# Autodesk Inventor assembly: GTPR Assembly - Laci
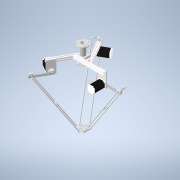
[picture p0: Inventor's stored thumbnail of the model, 180x180]
Saved by Autodesk Inventor 2021 (Build 250183000, 183)
## iProperties
Created: 2022-09-08
Part Number: GTPR Assembly - Laci
Document SubType Name: Assembly
Designer: Administrator
Title: GTPR Assembly - Laci v13
Author: Administrator
## Documents named in this file (17)
- C:\Git\PhD\Inventor\GTPR_toBeBuilt\GTPR Assembly - Laci.iam
- C:\Git\PhD\Inventor\GTPR_toBeBuilt\base frame.iam
- C:\Git\PhD\Inventor\GTPR_toBeBuilt\motor shaft clamp.ipt
- C:\Git\PhD\Inventor\GTPR_toBeBuilt\bosch b6 20x20 250 v1.ipt
- C:\Git\PhD\Inventor\GTPR_toBeBuilt\elbow keeper v1.ipt
- C:\Git\PhD\Inventor\GTPR_toBeBuilt\M8 Nut v5 v1.ipt
- C:\Git\PhD\Inventor\GTPR_toBeBuilt\inner.ipt
- C:\Git\PhD\Inventor\GTPR_toBeBuilt\outer.ipt
- C:\Git\PhD\Inventor\GTPR_toBeBuilt\lower arm 800.ipt
- C:\Git\PhD\Inventor\GTPR_toBeBuilt\WorkTriangleDisk.ipt
- C:\Git\PhD\Inventor\GTPR_toBeBuilt\workTrianglePc1.ipt
- C:\Users\szucs\Documents\Inventor\Content Center Files\R2021\en-US\AS 1420\AS 1420 - 1973 - M4 x 20.ipt
- C:\Users\szucs\Documents\Inventor\Content Center Files\R2021\en-US\AS 1237 (2.1)\AS 1237 - 4.ipt
- C:\Git\PhD\Inventor\GTPR_toBeBuilt\SKF_CAD_MODEL_SKF_W 624 R\AIS2021\SKF_W 624 R.iam
- C:\Git\PhD\Inventor\GTPR_toBeBuilt\rodFixerWasher.ipt
- C:\Git\PhD\Inventor\GTPR_toBeBuilt\rodFixer.ipt
- C:\Git\PhD\Inventor\GTPR_toBeBuilt\elbow clamp.ipt
## Components (95 placed, 16 different names)
1. base frame:1 [sub-assembly] — Flush:27, Mate:260, Flush:28, Mate:261, Flush:29, Mate:262, Angle:11, Angle:12, Angle:13
2. bosch b6 20x20 250 v1:2 — Mate:265, Flush:34, Flush:35, Flush:40, Flush:41, Mate:268
3. bosch b6 20x20 250 v1:3 — Flush:30, Flush:31, Mate:263, Flush:36, Flush:37, Mate:266
4. bosch b6 20x20 250 v1:4 — Mate:264, Flush:32, Flush:33, Flush:38, Mate:267, Flush:39
5. elbow keeper v1:1 — Mate:37, Mate:38, Flush:21, Flush:23, Mate:47, Mate:67, Mate:68, Mate:93, Mate:94, Mate:277
6. elbow keeper v1:2 — Mate:39, Mate:40, Flush:20, Flush:22, Mate:44, Mate:69, Mate:70, Mate:95, Mate:96, Mate:269
7. elbow keeper v1:3 — Mate:41, Mate:42, Flush:18, Flush:19, Mate:45, Mate:71, Mate:72, Mate:91, Mate:92, Mate:273
8. M8 Nut v5 v1:1 — Mate:38, Flush:21, Mate:196
9. M8 Nut v5 v1:2 — Mate:37, Flush:23, Mate:197
10. M8 Nut v5 v1:3 — Mate:39, Flush:20, Mate:198
11. M8 Nut v5 v1:4 — Mate:42, Flush:18, Mate:195
12. M8 Nut v5 v1:5 — Mate:40, Flush:22, Mate:199
13. M8 Nut v5 v1:6 — Mate:41, Flush:19, Mate:194
14. M8 Nut v5 v1:7 — Mate:44, Mate:270
15. M8 Nut v5 v1:9 — Mate:45, Mate:275
16. M8 Nut v5 v1:10 — Mate:47, Mate:279
17. inner:1 — Mate:72, Tangent:3, Mate:101, Mate:195
18. inner:2 — Mate:71, Tangent:4, Mate:102, Mate:194
19. inner:3 — Mate:70, Tangent:5, Mate:97, Mate:199
20. inner:4 — Mate:69, Tangent:6, Mate:98, Mate:198
21. inner:5 — Mate:68, Tangent:1, Mate:100, Mate:197
22. inner:6 — Mate:67, Tangent:2, Mate:99, Mate:196
23. outer:1 — Tangent:6, Mate:81, Mate:82
24. outer:2 — Tangent:5, Mate:79, Mate:80
25. outer:3 — Tangent:1, Mate:84, Mate:85
26. outer:4 — Tangent:2, Mate:83, Mate:86
27. outer:5 — Tangent:4, Mate:87, Mate:90
28. outer:6 — Tangent:3, Mate:88, Mate:89
29. lower arm 800:1 — Mate:79, Mate:80, Mate:123, Mate:124, Angle:10, Tangent:15, Mate:202
30. lower arm 800:2 — Mate:81, Mate:82, Mate:122, Mate:125, Angle:9, Mate:201, Tangent:14
31. lower arm 800:3 — Mate:84, Mate:85, Mate:119, Mate:158, Angle:8, Mate:259
32. lower arm 800:4 — Mate:83, Mate:86, Mate:120, Mate:121, Angle:7, Mate:258, Tangent:17
33. lower arm 800:5 — Mate:87, Mate:90, Mate:116, Mate:117, Angle:6, Mate:256, Tangent:16
34. lower arm 800:6 — Mate:88, Mate:89, Mate:115, Mate:118, Angle:5, Mate:257
35. M8 Nut v5 v1:13 — Mate:91, Mate:101, Mate:282
36. M8 Nut v5 v1:14 — Mate:96, Mate:98
37. M8 Nut v5 v1:15 — Mate:95, Mate:97, Mate:281
38. M8 Nut v5 v1:16 — Mate:93, Mate:100
39. M8 Nut v5 v1:17 — Mate:92, Mate:102
40. M8 Nut v5 v1:18 — Mate:94, Mate:99, Mate:283
41. inner:7 — Tangent:11, Mate:209, Mate:210
42. inner:8 — Tangent:12, Mate:207, Mate:208
43. inner:9 — Tangent:9, Mate:203, Mate:204
44. inner:10 — Tangent:10, Mate:205, Mate:206
45. inner:11 — Tangent:8, Mate:150, Mate:152
46. inner:12 — Tangent:13, Mate:151, Mate:153
47. outer:7 — Tangent:12, Mate:119, Mate:158, Angle:8
48. outer:8 — Tangent:11, Mate:120, Mate:121, Angle:7
49. outer:9 — Tangent:10, Mate:115, Mate:118, Angle:5
50. outer:10 — Tangent:9, Mate:116, Mate:117, Angle:6
51. outer:11 — Mate:123, Mate:124, Tangent:13, Angle:10
52. outer:12 — Tangent:8, Mate:122, Mate:125, Angle:9
53. WorkTriangleDisk:1 — Mate:284, Mate:285, Mate:286, Mate:287, Mate:288, Mate:289, Mate:290, Mate:291, Mate:292, Mate:293, Mate:294, Mate:295
54. workTrianglePc1:3 — Mate:207, Mate:208, Mate:209, Mate:210, Mate:286, Mate:287, Mate:292, Mate:293
55. workTrianglePc1:4 — Mate:203, Mate:204, Mate:205, Mate:206, Mate:285, Mate:288, Mate:289, Mate:294
56. workTrianglePc1:5 — Mate:150, Mate:151, Mate:152, Mate:153, Mate:284, Mate:290, Mate:291, Mate:295
57. AS 1420 - Metric M4 x 20:1 — Mate:171, Mate:174, Mate:177, Mate:178, Mate:200, Mate:202
58. AS 1237 (2.1) 4:3 — Mate:170, Mate:200, Tangent:15
59. SKF_W 624 R:1 [sub-assembly] — Mate:170, Mate:171, Mate:175, Mate:212, Mate:213
60. AS 1237 (2.1) 4:4 — Mate:174, Mate:175, Mate:176
61. rodFixerWasher:1 — Mate:176, Mate:177, Mate:178, Flush:24
62. AS 1420 - Metric M4 x 20:2 — Mate:183, Mate:184, Mate:186, Mate:188, Mate:189, Mate:201
63. AS 1237 (2.1) 4:5 — Mate:189, Tangent:14
64. SKF_W 624 R:2 [sub-assembly] — Mate:187, Mate:188, Mate:211
65. AS 1237 (2.1) 4:6 — Mate:185, Mate:186, Mate:187
66. rodFixerWasher:2 — Mate:183, Mate:184, Mate:185, Flush:24
67. rodFixer:1 — Mate:211, Mate:212, Mate:213
68. AS 1420 - Metric M4 x 20:3 — Mate:256
69. AS 1237 (2.1) 4:7 — Tangent:16
70. SKF_W 624 R:3 [sub-assembly]
71. AS 1237 (2.1) 4:8
72. rodFixerWasher:3
73. AS 1420 - Metric M4 x 20:4 — Mate:257
74. AS 1237 (2.1) 4:9
75. SKF_W 624 R:4 [sub-assembly]
76. AS 1237 (2.1) 4:10
77. rodFixerWasher:4
78. rodFixer:2
79. AS 1420 - Metric M4 x 20:5 — Mate:259
80. AS 1237 (2.1) 4:11
81. SKF_W 624 R:5 [sub-assembly]
82. AS 1237 (2.1) 4:12
83. rodFixerWasher:5
84. AS 1420 - Metric M4 x 20:6 — Mate:258
85. AS 1237 (2.1) 4:13 — Tangent:17
86. SKF_W 624 R:6 [sub-assembly]
87. AS 1237 (2.1) 4:14
88. rodFixerWasher:6
89. rodFixer:3
90. motor shaft clamp:1 — Flush:27, Mate:260, Mate:265, Flush:34, Flush:35, Angle:11
91. motor shaft clamp:2 — Flush:29, Mate:262, Flush:30, Flush:31, Mate:263, Angle:12
92. motor shaft clamp:3 — Flush:28, Mate:261, Mate:264, Flush:32, Flush:33, Angle:13
93. elbow clamp:1 — Flush:36, Flush:37, Mate:266, Mate:273, Mate:275, Mate:282
94. elbow clamp:2 — Flush:38, Mate:267, Flush:39, Mate:269, Mate:270, Mate:281
95. elbow clamp:3 — Flush:40, Flush:41, Mate:268, Mate:277, Mate:279, Mate:283
## Relationships (217: Mate 168, Flush 24, Tangent 16, Angle 9)
- Mate:37: elbow keeper v1:1 ↔ M8 Nut v5 v1:2
- Mate:38: elbow keeper v1:1 ↔ M8 Nut v5 v1:1
- Mate:39: elbow keeper v1:2 ↔ M8 Nut v5 v1:3
- Mate:40: elbow keeper v1:2 ↔ M8 Nut v5 v1:5
- Mate:41: elbow keeper v1:3 ↔ M8 Nut v5 v1:6
- Mate:42: elbow keeper v1:3 ↔ M8 Nut v5 v1:4
- Flush:18: elbow keeper v1:3 ↔ M8 Nut v5 v1:4
- Flush:19: elbow keeper v1:3 ↔ M8 Nut v5 v1:6
- Flush:20: elbow keeper v1:2 ↔ M8 Nut v5 v1:3
- Flush:21: elbow keeper v1:1 ↔ M8 Nut v5 v1:1
- Flush:22: elbow keeper v1:2 ↔ M8 Nut v5 v1:5
- Flush:23: elbow keeper v1:1 ↔ M8 Nut v5 v1:2
- Mate:44: elbow keeper v1:2 ↔ M8 Nut v5 v1:7
- Mate:45: elbow keeper v1:3 ↔ M8 Nut v5 v1:9
- Mate:47: elbow keeper v1:1 ↔ M8 Nut v5 v1:10
- Mate:67: elbow keeper v1:1 ↔ inner:6
- Mate:68: elbow keeper v1:1 ↔ inner:5
- Mate:69: elbow keeper v1:2 ↔ inner:4
- Mate:70: elbow keeper v1:2 ↔ inner:3
- Mate:71: elbow keeper v1:3 ↔ inner:2
- Mate:72: elbow keeper v1:3 ↔ inner:1
- Tangent:1: inner:5 ↔ outer:3
- Tangent:2: inner:6 ↔ outer:4
- Tangent:3: inner:1 ↔ outer:6
- Tangent:4: inner:2 ↔ outer:5
- Tangent:5: inner:3 ↔ outer:2
- Tangent:6: inner:4 ↔ outer:1
- Mate:79: outer:2 ↔ lower arm 800:1
- Mate:80: outer:2 ↔ lower arm 800:1
- Mate:81: outer:1 ↔ lower arm 800:2
- Mate:82: outer:1 ↔ lower arm 800:2
- Mate:83: outer:4 ↔ lower arm 800:4
- Mate:84: outer:3 ↔ lower arm 800:3
- Mate:85: outer:3 ↔ lower arm 800:3
- Mate:86: outer:4 ↔ lower arm 800:4
- Mate:87: outer:5 ↔ lower arm 800:5
- Mate:88: outer:6 ↔ lower arm 800:6
- Mate:89: outer:6 ↔ lower arm 800:6
- Mate:90: outer:5 ↔ lower arm 800:5
- Mate:91: elbow keeper v1:3 ↔ M8 Nut v5 v1:13
- Mate:92: elbow keeper v1:3 ↔ M8 Nut v5 v1:17
- Mate:93: elbow keeper v1:1 ↔ M8 Nut v5 v1:16
- Mate:94: elbow keeper v1:1 ↔ M8 Nut v5 v1:18
- Mate:95: elbow keeper v1:2 ↔ M8 Nut v5 v1:15
- Mate:96: elbow keeper v1:2 ↔ M8 Nut v5 v1:14
- Mate:97: inner:3 ↔ M8 Nut v5 v1:15
- Mate:98: inner:4 ↔ M8 Nut v5 v1:14
- Mate:99: inner:6 ↔ M8 Nut v5 v1:18
- Mate:100: inner:5 ↔ M8 Nut v5 v1:16
- Mate:101: inner:1 ↔ M8 Nut v5 v1:13
- Mate:102: inner:2 ↔ M8 Nut v5 v1:17
- Tangent:8: inner:11 ↔ outer:12
- Tangent:9: inner:9 ↔ outer:10
- Tangent:10: inner:10 ↔ outer:9
- Tangent:11: inner:7 ↔ outer:8
- Tangent:12: inner:8 ↔ outer:7
- Mate:115: lower arm 800:6 ↔ outer:9
- Mate:116: lower arm 800:5 ↔ outer:10
- Mate:117: lower arm 800:5 ↔ outer:10
- Mate:118: lower arm 800:6 ↔ outer:9
- Mate:119: lower arm 800:3 ↔ outer:7
- Mate:120: lower arm 800:4 ↔ outer:8
- Mate:121: lower arm 800:4 ↔ outer:8
- Mate:122: lower arm 800:2 ↔ outer:12
- Mate:123: lower arm 800:1 ↔ outer:11
- Mate:124: lower arm 800:1 ↔ outer:11
- Mate:125: lower arm 800:2 ↔ outer:12
- Tangent:13: inner:12 ↔ outer:11
- Mate:150: inner:11 ↔ workTrianglePc1:5
- Mate:151: inner:12 ↔ workTrianglePc1:5
- Mate:152: inner:11 ↔ workTrianglePc1:5
- Mate:153: inner:12 ↔ workTrianglePc1:5
- Mate:158: lower arm 800:3 ↔ outer:7
- Mate:170: AS 1237 (2.1) 4:3 ↔ SKF_W 624 R:1
- Mate:171: AS 1420 - Metric M4 x 20:1 ↔ SKF_W 624 R:1
- Mate:174: AS 1420 - Metric M4 x 20:1 ↔ AS 1237 (2.1) 4:4
- Mate:175: SKF_W 624 R:1 ↔ AS 1237 (2.1) 4:4
- Mate:176: AS 1237 (2.1) 4:4 ↔ rodFixerWasher:1
- Mate:177: AS 1420 - Metric M4 x 20:1 ↔ rodFixerWasher:1
- Mate:178: AS 1420 - Metric M4 x 20:1 ↔ rodFixerWasher:1
- [Mate]: AS 1237 (2.1) 4:5 ↔ SKF_W 624 R:2
- [Mate]: SKF_W 624 R:2 ↔ AS 1237 (2.1) 4:6
- [Mate]: AS 1237 (2.1) 4:6 ↔ rodFixerWasher:2
- Mate:183: AS 1420 - Metric M4 x 20:2 ↔ rodFixerWasher:2
- Mate:184: AS 1420 - Metric M4 x 20:2 ↔ rodFixerWasher:2
- Mate:185: AS 1237 (2.1) 4:6 ↔ rodFixerWasher:2
- Mate:186: AS 1420 - Metric M4 x 20:2 ↔ AS 1237 (2.1) 4:6
- Mate:187: SKF_W 624 R:2 ↔ AS 1237 (2.1) 4:6
- Mate:188: AS 1420 - Metric M4 x 20:2 ↔ SKF_W 624 R:2
- Mate:189: AS 1420 - Metric M4 x 20:2 ↔ AS 1237 (2.1) 4:5
- Angle:5 (90 deg): lower arm 800:6 ↔ outer:9
- Angle:6 (90 deg): lower arm 800:5 ↔ outer:10
- Angle:7 (90 deg): lower arm 800:4 ↔ outer:8
- Angle:8 (90 deg): lower arm 800:3 ↔ outer:7
- Angle:9 (90 deg): lower arm 800:2 ↔ outer:12
- Angle:10 (90 deg): lower arm 800:1 ↔ outer:11
- Mate:194: M8 Nut v5 v1:6 ↔ inner:2
- Mate:195: M8 Nut v5 v1:4 ↔ inner:1
- Mate:196: M8 Nut v5 v1:1 ↔ inner:6
- Mate:197: M8 Nut v5 v1:2 ↔ inner:5
- Mate:198: M8 Nut v5 v1:3 ↔ inner:4
- Mate:199: M8 Nut v5 v1:5 ↔ inner:3
- Mate:200: AS 1420 - Metric M4 x 20:1 ↔ AS 1237 (2.1) 4:3
- Mate:201: lower arm 800:2 ↔ AS 1420 - Metric M4 x 20:2
- Tangent:14: lower arm 800:2 ↔ AS 1237 (2.1) 4:5
- Tangent:15: lower arm 800:1 ↔ AS 1237 (2.1) 4:3
- Mate:202: lower arm 800:1 ↔ AS 1420 - Metric M4 x 20:1
- Mate:203: inner:9 ↔ workTrianglePc1:4
- Mate:204: inner:9 ↔ workTrianglePc1:4
- Mate:205: inner:10 ↔ workTrianglePc1:4
- Mate:206: inner:10 ↔ workTrianglePc1:4
- Mate:207: inner:8 ↔ workTrianglePc1:3
- Mate:208: inner:8 ↔ workTrianglePc1:3
- Mate:209: inner:7 ↔ workTrianglePc1:3
- Mate:210: inner:7 ↔ workTrianglePc1:3
- Flush:24: rodFixerWasher:1 ↔ rodFixerWasher:2
- Mate:211: SKF_W 624 R:2 ↔ rodFixer:1
- Mate:212: SKF_W 624 R:1 ↔ rodFixer:1
- Mate:213: SKF_W 624 R:1 ↔ rodFixer:1
- [Mate]: AS 1237 (2.1) 4:7 ↔ SKF_W 624 R:3
- [Mate]: AS 1420 - Metric M4 x 20:3 ↔ SKF_W 624 R:3
- [Mate]: AS 1420 - Metric M4 x 20:3 ↔ AS 1237 (2.1) 4:8
- [Mate]: SKF_W 624 R:3 ↔ AS 1237 (2.1) 4:8
- [Mate]: AS 1237 (2.1) 4:8 ↔ rodFixerWasher:3
- [Mate]: AS 1420 - Metric M4 x 20:3 ↔ rodFixerWasher:3
- [Mate]: AS 1420 - Metric M4 x 20:3 ↔ rodFixerWasher:3
- [Mate]: AS 1237 (2.1) 4:9 ↔ SKF_W 624 R:4
- [Mate]: SKF_W 624 R:4 ↔ AS 1237 (2.1) 4:10
- [Mate]: AS 1237 (2.1) 4:10 ↔ rodFixerWasher:4
- [Mate]: AS 1420 - Metric M4 x 20:4 ↔ rodFixerWasher:4
- [Mate]: AS 1420 - Metric M4 x 20:4 ↔ rodFixerWasher:4
- [Mate]: AS 1237 (2.1) 4:10 ↔ rodFixerWasher:4
- [Mate]: AS 1420 - Metric M4 x 20:4 ↔ AS 1237 (2.1) 4:10
- [Mate]: SKF_W 624 R:4 ↔ AS 1237 (2.1) 4:10
- [Mate]: AS 1420 - Metric M4 x 20:4 ↔ SKF_W 624 R:4
- [Mate]: AS 1420 - Metric M4 x 20:4 ↔ AS 1237 (2.1) 4:9
- [Mate]: AS 1420 - Metric M4 x 20:3 ↔ AS 1237 (2.1) 4:7
- [Flush]: rodFixerWasher:3 ↔ rodFixerWasher:4
- [Mate]: SKF_W 624 R:4 ↔ rodFixer:2
- [Mate]: SKF_W 624 R:3 ↔ rodFixer:2
- [Mate]: SKF_W 624 R:3 ↔ rodFixer:2
- [Mate]: AS 1237 (2.1) 4:11 ↔ SKF_W 624 R:5
- [Mate]: AS 1420 - Metric M4 x 20:5 ↔ SKF_W 624 R:5
- [Mate]: AS 1420 - Metric M4 x 20:5 ↔ AS 1237 (2.1) 4:12
- [Mate]: SKF_W 624 R:5 ↔ AS 1237 (2.1) 4:12
- [Mate]: AS 1237 (2.1) 4:12 ↔ rodFixerWasher:5
- [Mate]: AS 1420 - Metric M4 x 20:5 ↔ rodFixerWasher:5
- [Mate]: AS 1420 - Metric M4 x 20:5 ↔ rodFixerWasher:5
- [Mate]: AS 1237 (2.1) 4:13 ↔ SKF_W 624 R:6
- [Mate]: SKF_W 624 R:6 ↔ AS 1237 (2.1) 4:14
- [Mate]: AS 1237 (2.1) 4:14 ↔ rodFixerWasher:6
- [Mate]: AS 1420 - Metric M4 x 20:6 ↔ rodFixerWasher:6
- [Mate]: AS 1420 - Metric M4 x 20:6 ↔ rodFixerWasher:6
- [Mate]: AS 1237 (2.1) 4:14 ↔ rodFixerWasher:6
- [Mate]: AS 1420 - Metric M4 x 20:6 ↔ AS 1237 (2.1) 4:14
- [Mate]: SKF_W 624 R:6 ↔ AS 1237 (2.1) 4:14
- [Mate]: AS 1420 - Metric M4 x 20:6 ↔ SKF_W 624 R:6
- [Mate]: AS 1420 - Metric M4 x 20:6 ↔ AS 1237 (2.1) 4:13
- [Mate]: AS 1420 - Metric M4 x 20:5 ↔ AS 1237 (2.1) 4:11
- [Flush]: rodFixerWasher:5 ↔ rodFixerWasher:6
- [Mate]: SKF_W 624 R:6 ↔ rodFixer:3
- [Mate]: SKF_W 624 R:5 ↔ rodFixer:3
- [Mate]: SKF_W 624 R:5 ↔ rodFixer:3
- Mate:256: lower arm 800:5 ↔ AS 1420 - Metric M4 x 20:3
- Tangent:16: lower arm 800:5 ↔ AS 1237 (2.1) 4:7
- Mate:257: lower arm 800:6 ↔ AS 1420 - Metric M4 x 20:4
- Mate:258: lower arm 800:4 ↔ AS 1420 - Metric M4 x 20:6
- Tangent:17: lower arm 800:4 ↔ AS 1237 (2.1) 4:13
- Mate:259: lower arm 800:3 ↔ AS 1420 - Metric M4 x 20:5
- Flush:27: base frame:1 ↔ motor shaft clamp:1
- Mate:260: base frame:1 ↔ motor shaft clamp:1
- Flush:28: base frame:1 ↔ motor shaft clamp:3
- Mate:261: base frame:1 ↔ motor shaft clamp:3
- Flush:29: base frame:1 ↔ motor shaft clamp:2
- Mate:262: base frame:1 ↔ motor shaft clamp:2
- Flush:30: bosch b6 20x20 250 v1:3 ↔ motor shaft clamp:2
- Flush:31: bosch b6 20x20 250 v1:3 ↔ motor shaft clamp:2
- Mate:263: bosch b6 20x20 250 v1:3 ↔ motor shaft clamp:2
- Mate:264: bosch b6 20x20 250 v1:4 ↔ motor shaft clamp:3
- Flush:32: bosch b6 20x20 250 v1:4 ↔ motor shaft clamp:3
- Flush:33: bosch b6 20x20 250 v1:4 ↔ motor shaft clamp:3
- Mate:265: bosch b6 20x20 250 v1:2 ↔ motor shaft clamp:1
- Flush:34: bosch b6 20x20 250 v1:2 ↔ motor shaft clamp:1
- Flush:35: bosch b6 20x20 250 v1:2 ↔ motor shaft clamp:1
- Flush:36: bosch b6 20x20 250 v1:3 ↔ elbow clamp:1
- Flush:37: bosch b6 20x20 250 v1:3 ↔ elbow clamp:1
- Mate:266: bosch b6 20x20 250 v1:3 ↔ elbow clamp:1
- Flush:38: bosch b6 20x20 250 v1:4 ↔ elbow clamp:2
- Mate:267: bosch b6 20x20 250 v1:4 ↔ elbow clamp:2
- Flush:39: bosch b6 20x20 250 v1:4 ↔ elbow clamp:2
- Flush:40: bosch b6 20x20 250 v1:2 ↔ elbow clamp:3
- Flush:41: bosch b6 20x20 250 v1:2 ↔ elbow clamp:3
- Mate:268: bosch b6 20x20 250 v1:2 ↔ elbow clamp:3
- Mate:269: elbow keeper v1:2 ↔ elbow clamp:2
- Mate:270: M8 Nut v5 v1:7 ↔ elbow clamp:2
- Mate:273: elbow keeper v1:3 ↔ elbow clamp:1
- Mate:275: M8 Nut v5 v1:9 ↔ elbow clamp:1
- Mate:277: elbow keeper v1:1 ↔ elbow clamp:3
- Mate:279: M8 Nut v5 v1:10 ↔ elbow clamp:3
- Mate:281 (2.838 mm): M8 Nut v5 v1:15 ↔ elbow clamp:2
- Mate:282 (2.838 mm): M8 Nut v5 v1:13 ↔ elbow clamp:1
- Mate:283 (2.838 mm): M8 Nut v5 v1:18 ↔ elbow clamp:3
- Angle:11 (0 deg): base frame:1 ↔ motor shaft clamp:1
- Angle:12 (0 deg): base frame:1 ↔ motor shaft clamp:2
- Angle:13 (0 deg): base frame:1 ↔ motor shaft clamp:3
- Mate:284: WorkTriangleDisk:1 ↔ workTrianglePc1:5
- Mate:285: WorkTriangleDisk:1 ↔ workTrianglePc1:4
- Mate:286: WorkTriangleDisk:1 ↔ workTrianglePc1:3
- Mate:287: WorkTriangleDisk:1 ↔ workTrianglePc1:3
- Mate:288: WorkTriangleDisk:1 ↔ workTrianglePc1:4
- Mate:289: WorkTriangleDisk:1 ↔ workTrianglePc1:4
- Mate:290: WorkTriangleDisk:1 ↔ workTrianglePc1:5
- Mate:291: WorkTriangleDisk:1 ↔ workTrianglePc1:5
- Mate:292: WorkTriangleDisk:1 ↔ workTrianglePc1:3
- Mate:293: WorkTriangleDisk:1 ↔ workTrianglePc1:3
- Mate:294: WorkTriangleDisk:1 ↔ workTrianglePc1:4
- Mate:295: WorkTriangleDisk:1 ↔ workTrianglePc1:5
## Named parameters: d242_d230 = 0 mm, d243_d237 = 0 mm, d244_d238 = 0 mm, d290_d269 = 0 mm, d291_d286 = 0 mm, d292_d287 = 0 mm, d293_d288 = 0 mm, d294_d289 = 0 mm, d295_d242_d230 = 0 mm, d296_d243_d237 = 0 mm, d297_d244_d238 = 0 mm, d298_d245 = 0 mm, d299_d246 = 0 mm, d300_d247 = 0 mm, d301_d248 = 0 mm, d302_d249 = 0 mm, d303_d250 = 0 mm, d304_d251 = 0 mm, d305_d230 = 0 mm, d306_d231 = 0 mm, d307_d236 = 0 mm, d308_d237 = 0 mm, d309_d238 = 0 mm, d310_d239 = 0 mm, d311_d240 = 0 mm, d312_d269 = 0 mm, d313_d286 = 0 mm, d314_d287 = 0 mm, d315_d288 = 0 mm, d316_d289 = 0 mm, d317_d242_d230 = 0 mm, d318_d243_d237 = 0 mm, d319_d244_d238 = 0 mm, d320_d245 = 0 mm, d321_d246 = 0 mm, d322_d247 = 0 mm, d323_d248 = 0 mm, d324_d249 = 0 mm, d325_d250 = 0 mm, d326_d251 = 0 mm, d327_d230 = 0 mm, d328_d231 = 0 mm, d329_d236 = 0 mm, d330_d237 = 0 mm, d331_d238 = 0 mm, d332_d239 = 0 mm, d333_d240 = 0 mm
